# Autodesk Inventor assembly: basketleftservo
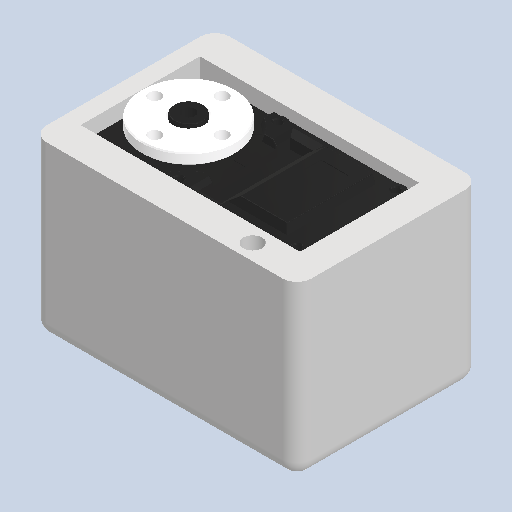
[picture p0: Inventor's stored thumbnail of the model, 512x512]
Saved by Autodesk Inventor 2025.3 (Build 293356000, 356)
## iProperties
Created: 2026-04-12
Part Number: basketleftservo
Document SubType Name: Assembly
Designer: ksawe
Author: ksawe
## Documents named in this file (3)
- C:\Users\ksawe\OneDrive\Pulpit\Exomy v1\wersja3\basketleftservo.iam
- C:\Users\ksawe\OneDrive\Pulpit\Exomy v1\wersja3\basketlewy.ipt
- C:\Users\ksawe\OneDrive\Pulpit\Exomy v1\wersja2\ST3215\ST3215\ST3215.ipt
## Components (2 placed, 2 different names)
1. basketlewy:1 — Mate:1, Mate:2
2. ST3215:1 — Mate:1, Mate:2
## Relationships (2: Mate 2)
- Mate:1: basketlewy:1 ↔ ST3215:1
- Mate:2: basketlewy:1 ↔ ST3215:1
